# Autodesk Inventor assembly: A2017_T3_03
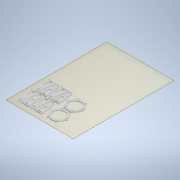
[picture p0: Inventor's stored thumbnail of the model, 180x180]
Saved by Autodesk Inventor 2020 (Build 240168000, 168)
## iProperties
Created: 2021-08-27
Part Number: A2017_T3_03
Document SubType Name: Assembly
Designer: Masato
Author: Masato
## Documents named in this file (4)
- C:\Inventor\SUSTAINA-OP\Cam\A2017_T3_03.iam
- C:\Inventor\SUSTAINA-OP\Cam\DisposableBoard.ipt
- C:\Inventor\SUSTAINA-OP\LowerBody\Leg_joint\Leg_joint_slider_frame.ipt
- C:\Inventor\SUSTAINA-OP\UpperBody\Trunk\CrossRollerBearing\Outer_flange.ipt
## Components (12 placed, 3 different names)
1. DisposableBoard:1 — メイト:2, メイト:1, フラッシュ:1, フラッシュ:2, フラッシュ:13, 角度:1, 正接:8, メイト:8, フラッシュ:14, メイト:9
2. Outer_flange:1 — フラッシュ:7
3. Leg_joint_slider_frame:1 — フラッシュ:6, フラッシュ:7, フラッシュ:13, メイト:5, 正接:3, メイト:8
4. Leg_joint_slider_frame:2 — フラッシュ:6, メイト:5, 正接:3, フラッシュ:14
5. Leg_joint_slider_frame:3
6. Leg_joint_slider_frame:4
7. Leg_joint_slider_frame:5
8. Leg_joint_slider_frame:6 — 正接:9
9. Leg_joint_slider_frame:7
10. Leg_joint_slider_frame:8
11. Outer_flange:2 — 角度:1, 正接:8, 正接:9, メイト:9
12. Outer_flange:3
## Component patterns: (4 elements, first: Leg_joint_slider_frame:1 + Leg_joint_slider_frame:2), (2 elements, first: Outer_flange:2)
## Relationships (15: Flush 6, Mate 5, Tangent 3, Angle 1)
- メイト:2 [Mate]: DisposableBoard:1
- メイト:1 [Mate]: DisposableBoard:1
- フラッシュ:1 [Flush]: DisposableBoard:1
- フラッシュ:2 [Flush]: DisposableBoard:1
- フラッシュ:6 [Flush]: Leg_joint_slider_frame:1 ↔ Leg_joint_slider_frame:2
- フラッシュ:7 [Flush]: Outer_flange:1 ↔ Leg_joint_slider_frame:1
- フラッシュ:13 [Flush] (2 mm): DisposableBoard:1 ↔ Leg_joint_slider_frame:1
- メイト:5 [Mate] (2.5 mm): Leg_joint_slider_frame:1 ↔ Leg_joint_slider_frame:2
- 正接:3 [Tangent]: Leg_joint_slider_frame:1 ↔ Leg_joint_slider_frame:2
- 角度:1 [Angle] (30 deg): DisposableBoard:1 ↔ Outer_flange:2
- 正接:8 [Tangent] (2 mm): DisposableBoard:1 ↔ Outer_flange:2
- メイト:8 [Mate]: DisposableBoard:1 ↔ Leg_joint_slider_frame:1
- フラッシュ:14 [Flush] (2 mm): DisposableBoard:1 ↔ Leg_joint_slider_frame:2
- 正接:9 [Tangent] (2.5 mm): Leg_joint_slider_frame:6 ↔ Outer_flange:2
- メイト:9 [Mate]: DisposableBoard:1 ↔ Outer_flange:2
